# Autodesk Inventor assembly: TS_V1_Fallmagazin_gesamt
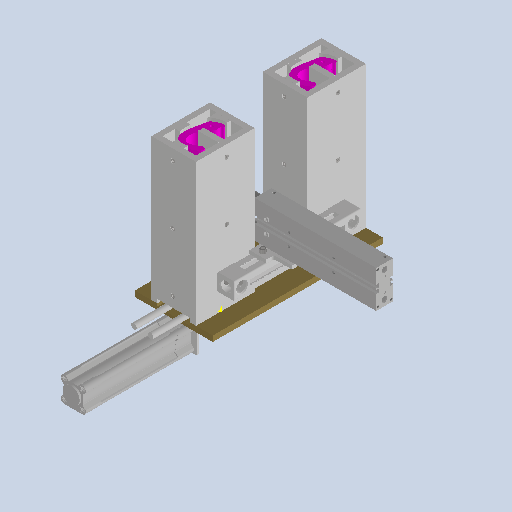
[picture p0: Inventor's stored thumbnail of the model, 512x512]
Saved by Autodesk Inventor 2025.1 (Build 291241000, 241)
## iProperties
Created: 2025-06-10
Part Number: TS_V1_Fallmagazin_gesamt
Document SubType Name: Assembly
Designer: tino
Author: tino
## Documents named in this file (29)
- C:\Users\Erik\Erik\Hochschule\3. Semester\CAD\CAD-Paspa\Useless Box\Eigene Bauteile\Fallmagazin\TS_V1_Fallmagazin_gesamt.iam
- C:\Users\Erik\Erik\Hochschule\3. Semester\CAD\CAD-Paspa\Useless Box\Eigene Bauteile\Fallmagazin\TS_V1_Fallmagazin_Boden_int.ipt
- C:\Users\Erik\Erik\Hochschule\3. Semester\CAD\CAD-Paspa\Useless Box\Eigene Bauteile\Fallmagazin\TS_V1_Fallmagazin_Wandung_int.ipt
- C:\Users\Erik\Erik\Hochschule\3. Semester\CAD\CAD-Paspa\Useless Box\Eigene Bauteile\Fallmagazin\TS_V1_Fallmagazin_Leitbleche_vorne_int.ipt
- C:\Users\Erik\Erik\Hochschule\3. Semester\CAD\CAD-Paspa\Useless Box\_Useless_Box\Finger.ipt
- C:\Users\Erik\Erik\Hochschule\3. Semester\CAD\CAD-Paspa\Useless Box\Eigene Bauteile\Fallmagazin\TS_V1_Fallmagazin_Schieber.iam
- C:\Users\Erik\Erik\Hochschule\3. Semester\CAD\CAD-Paspa\Useless Box\Kaufteile\Festo_Normzylinder_100\1376426 DSBC-32-100-PPVA-N3---(0).iam
- C:\Users\Erik\Erik\Hochschule\3. Semester\CAD\CAD-Paspa\Useless Box\Standart Bauteile\ISO 4762 - M4 x 12ISO.ipt
- C:\Users\Erik\Erik\Hochschule\3. Semester\CAD\CAD-Paspa\Useless Box\Standart Bauteile\ISO 4762 - M4 x 16ISO.ipt
- C:\Users\Erik\Erik\Hochschule\3. Semester\CAD\CAD-Paspa\Useless Box\Eigene Bauteile\Fallmagazin\TS_V1_Fallmagazin_Zylinderanbindung_int.ipt
- C:\Users\Erik\Erik\Hochschule\3. Semester\CAD\CAD-Paspa\Useless Box\Eigene Bauteile\Fallmagazin\TS_V1_Fallmagazin_Stopper_int.ipt
- C:\Users\Erik\Erik\Hochschule\3. Semester\CAD\CAD-Paspa\Useless Box\Eigene Bauteile\Fallmagazin\TS_V1_Fallmagazin_Zylinderhalter_int.ipt
- C:\Users\Erik\Erik\Hochschule\3. Semester\CAD\CAD-Paspa\Useless Box\Standart Bauteile\ISO 4762 - M5 x 8ISO.ipt
- C:\Users\Erik\Erik\Hochschule\3. Semester\CAD\CAD-Paspa\Useless Box\Standart Bauteile\ISO 4762 - M5 x 20ISO.ipt
- C:\Users\Erik\Erik\Hochschule\3. Semester\CAD\CAD-Paspa\Useless Box\Standart Bauteile\DIN EN ISO 2338 - 4 m6 x 10.ipt
- C:\Users\Erik\Erik\Hochschule\3. Semester\CAD\CAD-Paspa\Useless Box\Standart Bauteile\DIN 7991 - M5x12.ipt
- C:\Users\Erik\Erik\Hochschule\3. Semester\CAD\CAD-Paspa\Useless Box\Eigene Bauteile\Fallmagazin\TS_V1_Fallmagazin_Schieberanbindung_int.ipt
- C:\Users\Erik\Erik\Hochschule\3. Semester\CAD\CAD-Paspa\Useless Box\Eigene Bauteile\Fallmagazin\TS_V1_Fallmagazin_Verbindungsstange_int.ipt
- C:\Users\Erik\Erik\Hochschule\3. Semester\CAD\CAD-Paspa\Useless Box\Kaufteile\Festo_Fuehrungszylinder150_DFM_16\529120 DFM-16-150-B-P-A-KF---(0).iam
- C:\Users\Erik\Erik\Hochschule\3. Semester\CAD\CAD-Paspa\Useless Box\Kaufteile\DHRS-32-A - Kopie\AIS2024\1310164 DHRS-32-A---(0).iam
- C:\Users\Erik\Erik\Hochschule\3. Semester\CAD\CAD-Paspa\Useless Box\Eigene Bauteile\TS_Adapter_Greifer_int.ipt
- C:\Users\Erik\Erik\Hochschule\3. Semester\CAD\CAD-Paspa\Useless Box\Standart Bauteile\ISO 4762 - M4 x 10ISO.ipt
- C:\Users\Erik\Erik\Hochschule\3. Semester\CAD\CAD-Paspa\Useless Box\Eigene Bauteile\TS_Halterung_Fuehrungszylinder_int.ipt
- C:\Users\Erik\Erik\Hochschule\3. Semester\CAD\CAD-Paspa\Useless Box\Kaufteile\Rexroth_Profil+Winkel_30x30\Rexroth_30x30_Wuerfel\Rexroth_30x30_Wuerfel\Rexroth_30x30_Wuerfel.ipt
- C:\Users\Erik\Erik\Hochschule\3. Semester\CAD\CAD-Paspa\Useless Box\Kaufteile\Rexroth_Profil+Winkel_30x30\Rexroth_30x30_200_ext\Rexroth_30x30_200_ext\Rexroth_30x30_200_ext.ipt
- C:\Users\Erik\Erik\Hochschule\3. Semester\CAD\CAD-Paspa\Useless Box\Standart Bauteile\DIN 7991 - M8x16.ipt
- C:\Users\tino\Documents_VM\Inventor\Content Center Files\R2025\de-DE\DIN 934\DIN 934 - M5 x 0,8.ipt
- C:\Users\Erik\Erik\Hochschule\3. Semester\CAD\CAD-Paspa\Useless Box\Standart Bauteile\ISO 4762 - M6 x 12ISO.ipt
- C:\Users\Erik\Erik\Hochschule\3. Semester\CAD\CAD-Paspa\Useless Box\Kaufteile\Rexroth_Hammermuttern\Rexroth_Hammermutter_8_M6\Rexroth_Hammermutter_8_M6\Rexroth_Hammermutter_8_M6.ipt
## Components (189 placed, 28 different names)
1. TS_V1_Fallmagazin_Boden_int:1 — Mate:16, Mate:17, Mate:21, Mate:23, Mate:25, Mate:26, Mate:30, Mate:43, Mate:44, Mate:45, Mate:46, Flush:18, Mate:84, Mate:85, Mate:86, Mate:87, Mate:94, Mate:96, Mate:97, Flush:19, Flush:20, Mate:121
2. TS_V1_Fallmagazin_Wandung_int:2 — Mate:7, Mate:8, Flush:4, Angle:1, Angle:2, Mate:16, Mate:17, Mate:35, Mate:36, Mate:37, Mate:38, Mate:39, Mate:40, Mate:41, Mate:42, Angle:3, Mate:130
3. TS_V1_Fallmagazin_Leitbleche_vorne_int:1 — Mate:7, Mate:8, Flush:4, Tangent:2, Tangent:5, Flush:12
4. TS_V1_Fallmagazin_Schieber:1 [sub-assembly] — Mate:21, Mate:25, Mate:26, Mate:53, Mate:61, Mate:62, Mate:63, Mate:64, Mate:106, Tangent:6
5. TS_V1_Fallmagazin_Schieber:2 [sub-assembly] — Mate:23, Mate:30, Mate:65, Mate:66, Mate:67, Mate:101, Mate:103, Mate:107
6. 1376426 DSBC-32-100-PPVA-N3---(0):1 [sub-assembly] — Flush:18, Mate:68, Mate:69, Mate:92, Mate:93, Mate:99
7. TS_V1_Fallmagazin_Wandung_int:3 — Mate:45, Mate:46, Mate:47, Flush:14, Mate:48, Mate:132, Mate:137, Mate:138
8. TS_V1_Fallmagazin_Leitbleche_vorne_int:2 — Mate:47, Flush:14, Mate:48
9. TS_V1_Fallmagazin_Zylinderanbindung_int:1 — Mate:53, Mate:99, Angle:4, Mate:104, Mate:108, Mate:110, Mate:144
10. TS_V1_Fallmagazin_Stopper_int:1 — Mate:61, Mate:62, Angle:3
11. TS_V1_Fallmagazin_Stopper_int:2 — Mate:63, Mate:64
12. TS_V1_Fallmagazin_Stopper_int:3 — Mate:65, Flush:16, Mate:67
13. TS_V1_Fallmagazin_Stopper_int:4 — Mate:66, Flush:16
14. TS_V1_Fallmagazin_Zylinderhalter_int:1 — Mate:68, Mate:69, Mate:71, Mate:72, Mate:90, Mate:91, Mate:93, Mate:95, Mate:97
15. DIN 7991 M5x12:1 — Mate:106, Tangent:6, Mate:108
16. DIN 7991 M5x12:2 — Mate:101, Mate:107, Mate:109
17. TS_V1_Fallmagazin_Schieberanbindung_int:1 — Angle:4, Mate:103, Mate:105, Mate:109, Mate:142
18. TS_V1_Fallmagazin_Verbindungsstange_int:1 — Mate:104, Mate:105, Angle:5, Mate:110, Mate:141, Mate:143
19. 529120 DFM-16-150-B-P-A-KF---(0):1 [sub-assembly] — Flush:19, Angle:6, Flush:21, Mate:116, Mate:117, Mate:120, Mate:121, Mate:122, Mate:123, Mate:124, Angle:7, Angle:8
20. 1310164 DHRS-32-A---(0):1 [sub-assembly] — Flush:20, Flush:21, Mate:113, Mate:118, Mate:119
21. TS_Adapter_Greifer_int:1 — Mate:113, Mate:114, Mate:115, Mate:118, Mate:119, Mate:120
22. TS_Halterung_Fuehrungszylinder_int:1 — Mate:122, Mate:123, Mate:124, Mate:135, Mate:145, Mate:146, Mate:147, Mate:148, Mate:150, Mate:151, Mate:152
23. Rexroth_30x30_Wuerfel:1 — Mate:130, Mate:134, Flush:24, Flush:25, Mate:136, Tangent:7, Mate:139, Tangent:9
24. Rexroth_30x30_Wuerfel:2 — Mate:132, Mate:133, Flush:22, Flush:23, Mate:137, Tangent:8, Mate:140, Tangent:10
25. Rexroth_30x30_170_ext:1 — Mate:133, Flush:22, Flush:23, Mate:134, Flush:24, Flush:25, Mate:135, Tangent:11, Tangent:12
26. DIN 7991 M8x16:3 — Mate:136, Tangent:7
27. DIN 7991 M8x16:4 — Mate:138, Tangent:8
28. DIN 7991 M8x16:5 — Mate:139, Tangent:9
29. DIN 7991 M8x16:6 — Mate:140, Tangent:10
30. DIN 934 - ersetzt durch DIN EN 24032/28673/28674 M5:1 — Mate:141, Mate:142
31. DIN 934 - ersetzt durch DIN EN 24032/28673/28674 M5:2 — Mate:143, Mate:144
32. ISO 4762 - M6 x 12ISO:1 — Mate:147, Mate:148, Mate:149
33. Rexroth_Hammermutter_8_M6:1 — Angle:7, Tangent:11, Mate:149
34. Rexroth_Hammermutter_8_M6:2 — Angle:8, Tangent:12, Mate:150
35. ISO 4762 - M6 x 12ISO:2 — Mate:151, Mate:152
36. Finger:1 — Angle:1, Tangent:2, Tangent:5, Angle:2, Flush:12
37. Finger:2
38. Finger:3
39. Finger:4
40. Finger:5
41. Finger:6
42. Finger:7
43. Finger:8
44. Finger:9
45. Finger:10
46. Finger:11
47. Finger:12
48. Finger:13
49. Finger:14
50. Finger:15
51. Finger:16
52. Finger:17
53. Finger:18
54. Finger:19
55. Finger:20
56. Finger:21
57. Finger:22
58. Finger:23
59. Finger:24
60. Finger:25
61. Finger:26
62. Finger:27
63. Finger:28
64. Finger:29
65. Finger:30
66. Finger:31
67. Finger:32
68. Finger:33
69. Finger:34
70. Finger:35
71. Finger:36
72. Finger:37
73. Finger:38
74. Finger:39
75. Finger:40
76. Finger:41
77. Finger:42
78. Finger:43
79. Finger:44
80. Finger:45
81. Finger:46
82. Finger:47
83. Finger:48
84. Finger:49
85. Finger:50
86. Finger:51
87. Finger:52
88. Finger:53
89. Finger:54
90. Finger:55
91. Finger:56
92. Finger:57
93. Finger:58
94. Finger:59
95. Finger:60
96. Finger:61
97. Finger:62
98. Finger:63
99. Finger:64
100. Finger:65
101. Finger:66
102. Finger:67
103. Finger:68
104. Finger:69
105. Finger:70
106. Finger:71
107. Finger:72
108. Finger:73
109. Finger:74
110. Finger:75
111. Finger:76
112. Finger:77
113. Finger:78
114. Finger:79
115. Finger:80
116. Finger:81
117. Finger:82
118. Finger:83
119. Finger:84
120. Finger:85
121. Finger:86
122. Finger:87
123. Finger:88
124. Finger:89
125. Finger:90
126. Finger:91
127. Finger:92
128. Finger:93
129. Finger:94
130. Finger:95
131. Finger:96
132. Finger:97
133. Finger:98
134. ISO 4762 M5 x 8:1 — Mate:71, Mate:72, Mate:96
135. ISO 4762 M5 x 8:2
136. ISO 4762 M5 x 8:3 — Mate:94
137. ISO 4762 M5 x 8:4
138. ISO 4762 M5 x 20:1 — Mate:92, Mate:95
139. ISO 4762 M5 x 20:2 — Mate:91
140. ISO 4762 M5 x 20:3 — Mate:90
141. ISO 4762 M5 x 20:4
142. ISO 4762 M4 x 10:1 — Mate:114, Mate:115, Mate:116
143. ISO 4762 M4 x 10:2 — Mate:117
144. ISO 4762 M4 x 10:3
145. ISO 4762 M4 x 10:4
146. DIN EN ISO 2338 4 m6 x 10:1 — Mate:84, Mate:85
147. DIN EN ISO 2338 4 m6 x 10:2 — Mate:86, Mate:87
148. DIN EN ISO 2338 4 m6 x 10:3
149. DIN EN ISO 2338 4 m6 x 10:4
150. ISO 4762 M4 x 10:5 — Mate:145, Mate:146
151. ISO 4762 M4 x 10:6
152. ISO 4762 M4 x 10:7
153. ISO 4762 M4 x 10:8
154. ISO 4762 M4 x 12:1 — Mate:35, Mate:36
155. ISO 4762 M4 x 12:2
156. ISO 4762 M4 x 12:3
157. ISO 4762 M4 x 12:4 — Mate:37, Mate:38
158. ISO 4762 M4 x 12:5
159. ISO 4762 M4 x 12:6
160. ISO 4762 M4 x 12:7 — Mate:39, Mate:40
161. ISO 4762 M4 x 12:8
162. ISO 4762 M4 x 12:9
163. ISO 4762 M4 x 12:10 — Mate:41, Mate:42
164. ISO 4762 M4 x 12:11
165. ISO 4762 M4 x 12:12
166. ISO 4762 M4 x 16:1 — Mate:43, Mate:44
167. ISO 4762 M4 x 16:2
168. ISO 4762 M4 x 16:3
169. ISO 4762 M4 x 16:4
170. ISO 4762 M4 x 16:5
171. ISO 4762 M4 x 16:6
172. ISO 4762 M4 x 12:13
173. ISO 4762 M4 x 12:14
174. ISO 4762 M4 x 12:15
175. ISO 4762 M4 x 12:16
176. ISO 4762 M4 x 12:17
177. ISO 4762 M4 x 12:18
178. ISO 4762 M4 x 12:19
179. ISO 4762 M4 x 12:20
180. ISO 4762 M4 x 12:21
181. ISO 4762 M4 x 12:22
182. ISO 4762 M4 x 12:23
183. ISO 4762 M4 x 12:24
184. ISO 4762 M4 x 16:7
185. ISO 4762 M4 x 16:8
186. ISO 4762 M4 x 16:9
187. ISO 4762 M4 x 16:10
188. ISO 4762 M4 x 16:11
189. ISO 4762 M4 x 16:12
## Component patterns: (2 elements), (98 elements, first: Finger:1), (4 elements, first: ISO 4762 M5 x 8:1), (4 elements, first: ISO 4762 M5 x 20:1), (4 elements, first: ISO 4762 M4 x 10:1), (2 elements, first: DIN EN ISO 2338 4 m6 x 10:1 + DIN EN ISO 2338 4 m6 x 10:2), (4 elements, first: ISO 4762 M4 x 10:5), (3 elements, first: ISO 4762 M4 x 12:1), (3 elements, first: ISO 4762 M4 x 12:4), (3 elements, first: ISO 4762 M4 x 12:7), (3 elements, first: ISO 4762 M4 x 12:10), (6 elements, first: ISO 4762 M4 x 16:1), Komponentenanordnung 2:2 (3 elements), Komponentenanordnung 3:2 (3 elements), Komponentenanordnung 4:2 (3 elements), Komponentenanordnung 5:2 (3 elements), Komponentenanordnung 6:2 (6 elements)
## Relationships (120: Mate 91, Flush 12, Tangent 9, Angle 8)
- Mate:7: TS_V1_Fallmagazin_Wandung_int:2 ↔ TS_V1_Fallmagazin_Leitbleche_vorne_int:1
- Mate:8: TS_V1_Fallmagazin_Wandung_int:2 ↔ TS_V1_Fallmagazin_Leitbleche_vorne_int:1
- Flush:4: TS_V1_Fallmagazin_Wandung_int:2 ↔ TS_V1_Fallmagazin_Leitbleche_vorne_int:1
- Angle:1 (0 deg): TS_V1_Fallmagazin_Wandung_int:2 ↔ Finger:1
- Tangent:2: TS_V1_Fallmagazin_Leitbleche_vorne_int:1 ↔ Finger:1
- Tangent:5: TS_V1_Fallmagazin_Leitbleche_vorne_int:1 ↔ Finger:1
- Angle:2 (0 deg): TS_V1_Fallmagazin_Wandung_int:2 ↔ Finger:1
- Mate:16: TS_V1_Fallmagazin_Boden_int:1 ↔ TS_V1_Fallmagazin_Wandung_int:2
- Mate:17: TS_V1_Fallmagazin_Boden_int:1 ↔ TS_V1_Fallmagazin_Wandung_int:2
- Mate:21: TS_V1_Fallmagazin_Boden_int:1 ↔ TS_V1_Fallmagazin_Schieber:1
- Mate:23: TS_V1_Fallmagazin_Boden_int:1 ↔ TS_V1_Fallmagazin_Schieber:2
- Mate:25: TS_V1_Fallmagazin_Boden_int:1 ↔ TS_V1_Fallmagazin_Schieber:1
- Mate:26: TS_V1_Fallmagazin_Boden_int:1 ↔ TS_V1_Fallmagazin_Schieber:1
- Mate:30: TS_V1_Fallmagazin_Boden_int:1 ↔ TS_V1_Fallmagazin_Schieber:2
- Mate:35: TS_V1_Fallmagazin_Wandung_int:2 ↔ ISO 4762 M4 x 12:1
- Mate:36: TS_V1_Fallmagazin_Wandung_int:2 ↔ ISO 4762 M4 x 12:1
- Mate:37: TS_V1_Fallmagazin_Wandung_int:2 ↔ ISO 4762 M4 x 12:4
- Mate:38: TS_V1_Fallmagazin_Wandung_int:2 ↔ ISO 4762 M4 x 12:4
- Mate:39: TS_V1_Fallmagazin_Wandung_int:2 ↔ ISO 4762 M4 x 12:7
- Mate:40: TS_V1_Fallmagazin_Wandung_int:2 ↔ ISO 4762 M4 x 12:7
- Mate:41: TS_V1_Fallmagazin_Wandung_int:2 ↔ ISO 4762 M4 x 12:10
- Mate:42: TS_V1_Fallmagazin_Wandung_int:2 ↔ ISO 4762 M4 x 12:10
- Mate:43: TS_V1_Fallmagazin_Boden_int:1 ↔ ISO 4762 M4 x 16:1
- Mate:44: TS_V1_Fallmagazin_Boden_int:1 ↔ ISO 4762 M4 x 16:1
- Flush:12: TS_V1_Fallmagazin_Leitbleche_vorne_int:1 ↔ Finger:1
- Mate:45: TS_V1_Fallmagazin_Boden_int:1 ↔ TS_V1_Fallmagazin_Wandung_int:3
- Mate:46: TS_V1_Fallmagazin_Boden_int:1 ↔ TS_V1_Fallmagazin_Wandung_int:3
- Mate:47: TS_V1_Fallmagazin_Wandung_int:3 ↔ TS_V1_Fallmagazin_Leitbleche_vorne_int:2
- Flush:14: TS_V1_Fallmagazin_Wandung_int:3 ↔ TS_V1_Fallmagazin_Leitbleche_vorne_int:2
- Mate:48: TS_V1_Fallmagazin_Wandung_int:3 ↔ TS_V1_Fallmagazin_Leitbleche_vorne_int:2
- Mate:53: TS_V1_Fallmagazin_Schieber:1 ↔ TS_V1_Fallmagazin_Zylinderanbindung_int:1
- Mate:61: TS_V1_Fallmagazin_Schieber:1 ↔ TS_V1_Fallmagazin_Stopper_int:1
- Mate:62: TS_V1_Fallmagazin_Schieber:1 ↔ TS_V1_Fallmagazin_Stopper_int:1
- Mate:63: TS_V1_Fallmagazin_Schieber:1 ↔ TS_V1_Fallmagazin_Stopper_int:2
- Mate:64: TS_V1_Fallmagazin_Schieber:1 ↔ TS_V1_Fallmagazin_Stopper_int:2
- Mate:65: TS_V1_Fallmagazin_Schieber:2 ↔ TS_V1_Fallmagazin_Stopper_int:3
- Mate:66: TS_V1_Fallmagazin_Schieber:2 ↔ TS_V1_Fallmagazin_Stopper_int:4
- Flush:16: TS_V1_Fallmagazin_Stopper_int:3 ↔ TS_V1_Fallmagazin_Stopper_int:4
- Mate:67: TS_V1_Fallmagazin_Schieber:2 ↔ TS_V1_Fallmagazin_Stopper_int:3
- Flush:18: TS_V1_Fallmagazin_Boden_int:1 ↔ 1376426 DSBC-32-100-PPVA-N3---(0):1
- Mate:68: 1376426 DSBC-32-100-PPVA-N3---(0):1 ↔ TS_V1_Fallmagazin_Zylinderhalter_int:1
- Mate:69: 1376426 DSBC-32-100-PPVA-N3---(0):1 ↔ TS_V1_Fallmagazin_Zylinderhalter_int:1
- Mate:71: TS_V1_Fallmagazin_Zylinderhalter_int:1 ↔ ISO 4762 M5 x 8:1
- Mate:72: TS_V1_Fallmagazin_Zylinderhalter_int:1 ↔ ISO 4762 M5 x 8:1
- Mate:84: TS_V1_Fallmagazin_Boden_int:1 ↔ DIN EN ISO 2338 4 m6 x 10:1
- Mate:85 (0.5 mm): TS_V1_Fallmagazin_Boden_int:1 ↔ DIN EN ISO 2338 4 m6 x 10:1
- Mate:86: TS_V1_Fallmagazin_Boden_int:1 ↔ DIN EN ISO 2338 4 m6 x 10:2
- Mate:87 (1 mm): TS_V1_Fallmagazin_Boden_int:1 ↔ DIN EN ISO 2338 4 m6 x 10:2
- Angle:3 (0 deg): TS_V1_Fallmagazin_Wandung_int:2 ↔ TS_V1_Fallmagazin_Stopper_int:1
- Mate:90: TS_V1_Fallmagazin_Zylinderhalter_int:1 ↔ ISO 4762 M5 x 20:3
- Mate:91: TS_V1_Fallmagazin_Zylinderhalter_int:1 ↔ ISO 4762 M5 x 20:2
- Mate:92: 1376426 DSBC-32-100-PPVA-N3---(0):1 ↔ ISO 4762 M5 x 20:1
- Mate:93: 1376426 DSBC-32-100-PPVA-N3---(0):1 ↔ TS_V1_Fallmagazin_Zylinderhalter_int:1
- Mate:94: TS_V1_Fallmagazin_Boden_int:1 ↔ ISO 4762 M5 x 8:3
- Mate:95: TS_V1_Fallmagazin_Zylinderhalter_int:1 ↔ ISO 4762 M5 x 20:1
- Mate:96: TS_V1_Fallmagazin_Boden_int:1 ↔ ISO 4762 M5 x 8:1
- Mate:97: TS_V1_Fallmagazin_Boden_int:1 ↔ TS_V1_Fallmagazin_Zylinderhalter_int:1
- Mate:99: 1376426 DSBC-32-100-PPVA-N3---(0):1 ↔ TS_V1_Fallmagazin_Zylinderanbindung_int:1
- Mate:101: TS_V1_Fallmagazin_Schieber:2 ↔ DIN 7991 M5x12:2
- Angle:4 (180 deg): TS_V1_Fallmagazin_Zylinderanbindung_int:1 ↔ TS_V1_Fallmagazin_Schieberanbindung_int:1
- Mate:103: TS_V1_Fallmagazin_Schieber:2 ↔ TS_V1_Fallmagazin_Schieberanbindung_int:1
- Mate:104: TS_V1_Fallmagazin_Zylinderanbindung_int:1 ↔ TS_V1_Fallmagazin_Verbindungsstange_int:1
- Mate:105 (-10 mm): TS_V1_Fallmagazin_Schieberanbindung_int:1 ↔ TS_V1_Fallmagazin_Verbindungsstange_int:1
- Angle:5 (0 deg): TS_V1_Fallmagazin_Verbindungsstange_int:1
- Mate:106: TS_V1_Fallmagazin_Schieber:1 ↔ DIN 7991 M5x12:1
- Tangent:6: TS_V1_Fallmagazin_Schieber:1 ↔ DIN 7991 M5x12:1
- Mate:107: TS_V1_Fallmagazin_Schieber:2 ↔ DIN 7991 M5x12:2
- Mate:108: TS_V1_Fallmagazin_Zylinderanbindung_int:1 ↔ DIN 7991 M5x12:1
- Mate:109: DIN 7991 M5x12:2 ↔ TS_V1_Fallmagazin_Schieberanbindung_int:1
- Mate:110 (-10 mm): TS_V1_Fallmagazin_Zylinderanbindung_int:1 ↔ TS_V1_Fallmagazin_Verbindungsstange_int:1
- Flush:19 (22.694 mm): TS_V1_Fallmagazin_Boden_int:1 ↔ 529120 DFM-16-150-B-P-A-KF---(0):1
- Angle:6 (0 deg): 529120 DFM-16-150-B-P-A-KF---(0):1
- Flush:20 (-135 mm): TS_V1_Fallmagazin_Boden_int:1 ↔ 1310164 DHRS-32-A---(0):1
- Flush:21: 529120 DFM-16-150-B-P-A-KF---(0):1 ↔ 1310164 DHRS-32-A---(0):1
- Mate:113: 1310164 DHRS-32-A---(0):1 ↔ TS_Adapter_Greifer_int:1
- Mate:114: TS_Adapter_Greifer_int:1 ↔ ISO 4762 M4 x 10:1
- Mate:115: TS_Adapter_Greifer_int:1 ↔ ISO 4762 M4 x 10:1
- Mate:116: 529120 DFM-16-150-B-P-A-KF---(0):1 ↔ ISO 4762 M4 x 10:1
- Mate:117: 529120 DFM-16-150-B-P-A-KF---(0):1 ↔ ISO 4762 M4 x 10:2
- Mate:118: 1310164 DHRS-32-A---(0):1 ↔ TS_Adapter_Greifer_int:1
- Mate:119: 1310164 DHRS-32-A---(0):1 ↔ TS_Adapter_Greifer_int:1
- Mate:120: 529120 DFM-16-150-B-P-A-KF---(0):1 ↔ TS_Adapter_Greifer_int:1
- Mate:121 (30.575 mm): TS_V1_Fallmagazin_Boden_int:1 ↔ 529120 DFM-16-150-B-P-A-KF---(0):1
- Mate:122: 529120 DFM-16-150-B-P-A-KF---(0):1 ↔ TS_Halterung_Fuehrungszylinder_int:1
- Mate:123: 529120 DFM-16-150-B-P-A-KF---(0):1 ↔ TS_Halterung_Fuehrungszylinder_int:1
- Mate:124: 529120 DFM-16-150-B-P-A-KF---(0):1 ↔ TS_Halterung_Fuehrungszylinder_int:1
- Mate:130: TS_V1_Fallmagazin_Wandung_int:2 ↔ Rexroth_30x30_Wuerfel:1
- Mate:132: TS_V1_Fallmagazin_Wandung_int:3 ↔ Rexroth_30x30_Wuerfel:2
- Mate:133: Rexroth_30x30_Wuerfel:2 ↔ Rexroth_30x30_170_ext:1
- Flush:22: Rexroth_30x30_Wuerfel:2 ↔ Rexroth_30x30_170_ext:1
- Flush:23: Rexroth_30x30_Wuerfel:2 ↔ Rexroth_30x30_170_ext:1
- Mate:134: Rexroth_30x30_Wuerfel:1 ↔ Rexroth_30x30_170_ext:1
- Flush:24: Rexroth_30x30_Wuerfel:1 ↔ Rexroth_30x30_170_ext:1
- Flush:25: Rexroth_30x30_Wuerfel:1 ↔ Rexroth_30x30_170_ext:1
- Mate:135: TS_Halterung_Fuehrungszylinder_int:1 ↔ Rexroth_30x30_170_ext:1
- Mate:136: Rexroth_30x30_Wuerfel:1 ↔ DIN 7991 M8x16:3
- Tangent:7: Rexroth_30x30_Wuerfel:1 ↔ DIN 7991 M8x16:3
- Mate:137: TS_V1_Fallmagazin_Wandung_int:3 ↔ Rexroth_30x30_Wuerfel:2
- Mate:138: TS_V1_Fallmagazin_Wandung_int:3 ↔ DIN 7991 M8x16:4
- Tangent:8: Rexroth_30x30_Wuerfel:2 ↔ DIN 7991 M8x16:4
- Mate:139: Rexroth_30x30_Wuerfel:1 ↔ DIN 7991 M8x16:5
- Tangent:9: Rexroth_30x30_Wuerfel:1 ↔ DIN 7991 M8x16:5
- Mate:140: Rexroth_30x30_Wuerfel:2 ↔ DIN 7991 M8x16:6
- Tangent:10: Rexroth_30x30_Wuerfel:2 ↔ DIN 7991 M8x16:6
- Mate:141: TS_V1_Fallmagazin_Verbindungsstange_int:1 ↔ DIN 934 - ersetzt durch DIN EN 24032/28673/28674 M5:1
- Mate:142: TS_V1_Fallmagazin_Schieberanbindung_int:1 ↔ DIN 934 - ersetzt durch DIN EN 24032/28673/28674 M5:1
- Mate:143: TS_V1_Fallmagazin_Verbindungsstange_int:1 ↔ DIN 934 - ersetzt durch DIN EN 24032/28673/28674 M5:2
- Mate:144: TS_V1_Fallmagazin_Zylinderanbindung_int:1 ↔ DIN 934 - ersetzt durch DIN EN 24032/28673/28674 M5:2
- Mate:145: TS_Halterung_Fuehrungszylinder_int:1 ↔ ISO 4762 M4 x 10:5
- Mate:146: TS_Halterung_Fuehrungszylinder_int:1 ↔ ISO 4762 M4 x 10:5
- Mate:147: TS_Halterung_Fuehrungszylinder_int:1 ↔ ISO 4762 - M6 x 12ISO:1
- Mate:148: TS_Halterung_Fuehrungszylinder_int:1 ↔ ISO 4762 - M6 x 12ISO:1
- Angle:7 (180 deg): 529120 DFM-16-150-B-P-A-KF---(0):1 ↔ Rexroth_Hammermutter_8_M6:1
- Tangent:11: Rexroth_30x30_170_ext:1 ↔ Rexroth_Hammermutter_8_M6:1
- Mate:149: ISO 4762 - M6 x 12ISO:1 ↔ Rexroth_Hammermutter_8_M6:1
- Angle:8 (0 deg): 529120 DFM-16-150-B-P-A-KF---(0):1 ↔ Rexroth_Hammermutter_8_M6:2
- Tangent:12: Rexroth_30x30_170_ext:1 ↔ Rexroth_Hammermutter_8_M6:2
- Mate:150: TS_Halterung_Fuehrungszylinder_int:1 ↔ Rexroth_Hammermutter_8_M6:2
- Mate:151: TS_Halterung_Fuehrungszylinder_int:1 ↔ ISO 4762 - M6 x 12ISO:2
- Mate:152: TS_Halterung_Fuehrungszylinder_int:1 ↔ ISO 4762 - M6 x 12ISO:2
## Named parameters: Magazin_Hoehe = 255 mm, Abstand_Schrauben_vert = 105 mm, Abstand_Rand = 45 mm, Anbindung_Zylinder = 16.4 mm
